# Autodesk Inventor assembly: Основание с колесом нижнего редуктора
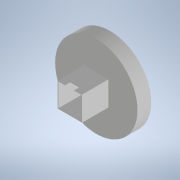
[picture p0: Inventor's stored thumbnail of the model, 180x180]
Saved by Autodesk Inventor 2021 (Build 250183000, 183)
## iProperties
Created: 2021-07-29
Part Number: Основание с колесом нижнего редуктора
Document SubType Name: Assembly
Designer: User
Author: User
## Documents named in this file (3)
- D:\INVENTOR\Аватар\3D-моделирование\1.2 ось доп. модели\Основание с колесом нижнего редуктора\Основание с колесом нижнего редуктора.iam
- D:\INVENTOR\Аватар\3D-моделирование\1.2 ось доп. модели\Основание с колесом нижнего редуктора\Основание.ipt
- D:\INVENTOR\Аватар\3D-моделирование\1.2 ось доп. модели\Основание с колесом нижнего редуктора\Цилиндрическое зубчатое зацепление21.ipt
## Components (2 placed, 2 different names)
1. Основание:1 — Заподлицо:1, Касательность:1
2. Цилиндрическое зубчатое зацепление2:1 — Заподлицо:1, Касательность:1
## Relationships (2: Flush 1, Tangent 1)
- Заподлицо:1 [Flush]: Основание:1 ↔ Цилиндрическое зубчатое зацепление2:1
- Касательность:1 [Tangent]: Основание:1 ↔ Цилиндрическое зубчатое зацепление2:1
